# Autodesk Inventor assembly: Engine Assembly
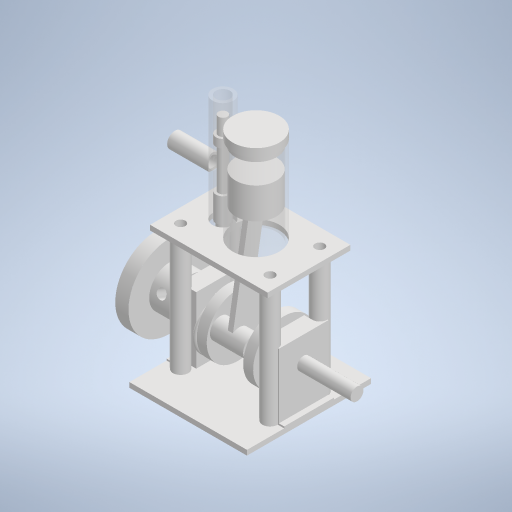
[picture p0: Inventor's stored thumbnail of the model, 512x512]
Saved by Autodesk Inventor 2023 (Build 270158000, 158)
## iProperties
Created: 2023-02-13
Part Number: Engine Assembly
Document SubType Name: Assembly
Designer: tommy
Author: tommy
## Documents named in this file (10)
- C:\Users\tommy\Documents\Repositories\Steam-Engine\Les Proper Steam Engine\CAD\Engine Assembly.iam
- C:\Users\tommy\Documents\Repositories\Steam-Engine\Les Proper Steam Engine\CAD\Base Bottom.ipt
- C:\Users\tommy\Documents\Repositories\Steam-Engine\Les Proper Steam Engine\CAD\Frame Post.ipt
- C:\Users\tommy\Documents\Repositories\Steam-Engine\Les Proper Steam Engine\CAD\Cylinder Assembly.iam
- C:\Users\tommy\Documents\Repositories\Steam-Engine\Les Proper Steam Engine\CAD\Piston Assembly.iam
- C:\Users\tommy\Documents\Repositories\Steam-Engine\Les Proper Steam Engine\CAD\Connecting Rod Assembly.iam
- C:\Users\tommy\Documents\Repositories\Steam-Engine\Les Proper Steam Engine\CAD\Valve.ipt
- C:\Users\tommy\Documents\Repositories\Steam-Engine\Les Proper Steam Engine\CAD\Crankshaft Assembly.iam
- C:\Users\tommy\Documents\Repositories\Steam-Engine\Les Proper Steam Engine\CAD\Valve Rod.ipt
- C:\Users\tommy\Documents\Repositories\Steam-Engine\Les Proper Steam Engine\CAD\Ease of Model Bearing.ipt
## Components (13 placed, 9 different names)
1. Connecting Rod Assembly:1 [sub-assembly] — Mate:19, Mate:20, Mate:21, Mate:22
2. Crankshaft Assembly:1 [sub-assembly] — Mate:18, Mate:19, Mate:20, Mate:24
3. Cylinder Assembly:1 [sub-assembly] — Mate:1, Mate:2, Mate:3, Mate:4, Mate:5, Mate:6, Mate:7, Mate:8, Mate:16, Flush:3, Mate:23
4. Ease of Model Bearing:1 — Flush:2, Mate:14, Mate:15
5. Piston Assembly:1 [sub-assembly] — Mate:21, Mate:22, Flush:3, Mate:23
6. Valve Rod:1 — Mate:17, Mate:18
7. Valve:1 — Mate:16, Mate:17
8. Ease of Model Bearing:2 — Mate:12, Flush:1, Mate:13, Mate:24
9. Base Bottom:1 — Mate:9, Mate:10, Mate:11, Mate:12, Flush:1, Flush:2, Mate:15
10. Frame Post:1 — Mate:1, Mate:7
11. Frame Post:2 — Mate:2, Mate:5
12. Frame Post:3 — Mate:3, Mate:6, Mate:11, Mate:13
13. Frame Post:4 — Mate:4, Mate:8, Mate:9, Mate:10, Mate:14
## Relationships (27: Mate 24, Flush 3)
- Mate:1: Cylinder Assembly:1 ↔ Frame Post:1
- Mate:2: Cylinder Assembly:1 ↔ Frame Post:2
- Mate:3: Cylinder Assembly:1 ↔ Frame Post:3
- Mate:4: Cylinder Assembly:1 ↔ Frame Post:4
- Mate:5: Cylinder Assembly:1 ↔ Frame Post:2
- Mate:6: Cylinder Assembly:1 ↔ Frame Post:3
- Mate:7: Cylinder Assembly:1 ↔ Frame Post:1
- Mate:8: Cylinder Assembly:1 ↔ Frame Post:4
- Mate:9: Base Bottom:1 ↔ Frame Post:4
- Mate:10: Base Bottom:1 ↔ Frame Post:4
- Mate:11: Base Bottom:1 ↔ Frame Post:3
- Mate:12: Ease of Model Bearing:2 ↔ Base Bottom:1
- Flush:1: Ease of Model Bearing:2 ↔ Base Bottom:1
- Mate:13: Ease of Model Bearing:2 ↔ Frame Post:3
- Flush:2: Ease of Model Bearing:1 ↔ Base Bottom:1
- Mate:14: Ease of Model Bearing:1 ↔ Frame Post:4
- Mate:15: Ease of Model Bearing:1 ↔ Base Bottom:1
- Mate:16: Cylinder Assembly:1 ↔ Valve:1
- Mate:17: Valve Rod:1 ↔ Valve:1
- Mate:18: Crankshaft Assembly:1 ↔ Valve Rod:1
- Mate:19: Connecting Rod Assembly:1 ↔ Crankshaft Assembly:1
- Mate:20 (0.254 mm): Connecting Rod Assembly:1 ↔ Crankshaft Assembly:1
- Mate:21: Connecting Rod Assembly:1 ↔ Piston Assembly:1
- Mate:22: Connecting Rod Assembly:1 ↔ Piston Assembly:1
- Flush:3: Cylinder Assembly:1 ↔ Piston Assembly:1
- Mate:23: Cylinder Assembly:1 ↔ Piston Assembly:1
- Mate:24: Crankshaft Assembly:1 ↔ Ease of Model Bearing:2
